# Autodesk Inventor assembly: Car_Assembly
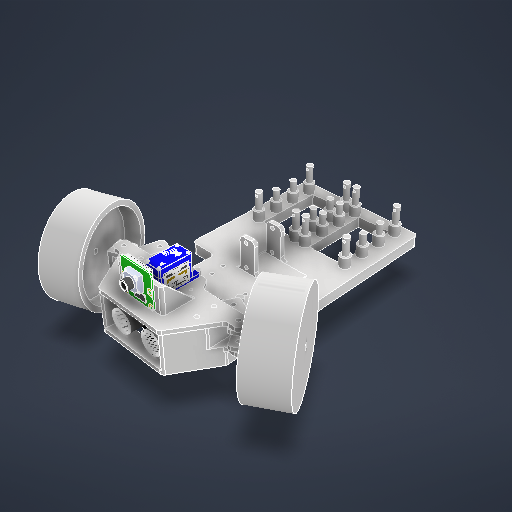
[picture p0: Inventor's stored thumbnail of the model, 512x512]
Saved by Autodesk Inventor 2025 (Build 290162000, 162)
## iProperties
Created: 2024-05-24
Part Number: Car_Assembly
Document SubType Name: Assembly
Designer: Garfieldcmix
Author: Garfieldcmix
## Documents named in this file (30)
- C:\Users\chaya\Desktop\WRO-2024-CAD\Inventor\Car_Assembly.iam
- C:\Users\chaya\Desktop\WRO-2024-CAD\Inventor\SG90 - Micro Servo 9g - Tower Pro\SG90 - Micro Servo 9g - Tower Pro.iam
- C:\Users\chaya\Desktop\WRO-2024-CAD\Inventor\Front_Bridge.ipt
- C:\Users\chaya\Desktop\WRO-2024-CAD\Inventor\Front_Wheel_Anchor.ipt
- C:\Users\chaya\Desktop\WRO-2024-CAD\Inventor\Front_Wheel_Anchor_MIR.ipt
- C:\Users\chaya\Desktop\WRO-2024-CAD\Inventor\Wheel.ipt
- C:\Users\chaya\Desktop\WRO-2024-CAD\Inventor\Wheel_MIR.ipt
- C:\Users\chaya\Desktop\WRO-2024-CAD\Inventor\Pi camera module3\Pi camera module3.ipt
- C:\Users\chaya\Desktop\WRO-2024-CAD\Inventor\4519 DkStone Technic Axle 3\4519 DkStone Technic Axle 3.ipt
- C:\Users\chaya\Desktop\WRO-2024-CAD\Inventor\Lego Beam Fram 5x7 (64179)\Lego Beam Fram 5x7 (64179).ipt
- C:\Users\chaya\Desktop\WRO-2024-CAD\Inventor\TT Motor\TT Motor.ipt
- C:\Users\chaya\Desktop\WRO-2024-CAD\Inventor\Lower_Chassis.ipt
- C:\Users\chaya\Desktop\WRO-2024-CAD\Inventor\Motor_Lego_Axle_Connector.ipt
- C:\Users\chaya\Desktop\WRO-2024-CAD\Inventor\Wheel_Lego_Axle_Connector.ipt
- C:\Users\chaya\Desktop\WRO-2024-CAD\Inventor\Front_Bridge_2.ipt
- C:\Users\chaya\Desktop\WRO-2024-CAD\Inventor\Servo_Steering_Linkage.ipt
- C:\Users\chaya\Desktop\WRO-2024-CAD\Inventor\hc-sr04\hc-sr04.iam
- C:\Users\chaya\Desktop\WRO-2024-CAD\Inventor\Lego_Frame_Holder.ipt
- C:\Users\chaya\Desktop\WRO-2024-CAD\Inventor\Lego_Frame_Holder_Extra.ipt
- C:\Users\chaya\Desktop\WRO-2024-CAD\Inventor\Lego_Frame_Holder_Extra_2.ipt
- C:\Users\chaya\Desktop\WRO-2024-CAD\Inventor\1.5_base.ipt
- C:\Users\chaya\Desktop\WRO-2024-CAD\Inventor\18650 2-WAY v5\18650 2-WAY v5.iam
- C:\Users\chaya\Desktop\WRO-2024-CAD\Inventor\MAKER-DRIVE\MAKER-DRIVE.iam
- C:\Users\chaya\Desktop\WRO-2024-CAD\Inventor\MPU_6050\MPU_6050.iam
- C:\Users\chaya\Desktop\WRO-2024-CAD\Inventor\RASPBERRY_PI_5\RASPBERRY_PI_5.iam
- C:\Users\chaya\Desktop\WRO-2024-CAD\Inventor\arduino nano\arduino nano.iam
- C:\Users\chaya\Desktop\WRO-2024-CAD\Inventor\Lego-Frame-Holder-Extra-Extra.ipt
- C:\Users\chaya\Desktop\WRO-2024-CAD\Inventor\SG90_Horn.ipt
- C:\Users\chaya\Desktop\WRO-2024-CAD\Inventor\2_Base.ipt
- C:\Users\chaya\Desktop\WRO-2024-CAD\Inventor\Wheel_Lego_Axle_Connector_2.ipt
## Components (54 placed, 37 different names)
1. Pi camera module3:1 — Mate:73, Mate:72, Mate:74
2. hc-sr04:1 [sub-assembly] — Mate:92, Mate:93, Mate:94
3. SG90_Servo [sub-assembly] — Mate:1, Mate:16, Mate:69, Mate:137, Mate:138
4. SG90_Horn:1 — Mate:137, Mate:138, Mate:139, Mate:141, Mate:201
5. Left_Servo_Steering_Linkage — Mate:85, Mate:83, Mate:139, Mate:141, Mate:202
6. Right_Servo_Steering_Linkage — Mate:199, Mate:200, Mate:201, Mate:202
7. Front_Bridge:1 — Mate:38, Mate:39, Mate:40, Mate:41, Mate:42, Mate:66, Mate:67, Mate:68, Mate:75, Mate:76, Mate:79, Mate:80, Angle:1, Mate:92, Mate:93, Mate:94
8. Front_Bridge_2:1 — Mate:66, Mate:67, Mate:68, Mate:69, Mate:73, Mate:72, Mate:74, Mate:1, Mate:16
9. Left_Front_Wheel_Anchor — Mate:75, Mate:76, Mate:77, Mate:78, Mate:85, Mate:83, Angle:1
10. Left_Front_Wheel — Mate:77, Mate:78
11. Right_Front_Wheel_Anchor — Mate:79, Mate:80, Mate:81, Mate:82, Mate:199, Mate:200
12. Right_Front_Wheel — Mate:81, Mate:82
13. Lower_Chassis:1 — Mate:38, Mate:39, Mate:40, Mate:41, Mate:42, Mate:43, Mate:44, Mate:45, Mate:46, Mate:47, Mate:48, Mate:57, Mate:91, Mate:96, Mate:97, Mate:98, Mate:100, Mate:101, Mate:103, Mate:104, Mate:106, Mate:107, Mate:109, Mate:110, Mate:112, Mate:113, Mate:115, Mate:116, Mate:118, Mate:119, Mate:120, Mate:121, Mate:122, Mate:123, Mate:124
14. Left_Lego_Beam_Frame — Mate:37, Mate:43, Mate:44, Mate:45, Mate:50, Mate:55, Mate:60, Mate:102, Mate:105, Mate:108, Mate:117
15. Lego_Driving_Shaft_Axle — Mate:50, Mate:53, Mate:54
16. TT Motor:1 — Mate:51, Mate:52, Mate:57, Mate:91
17. Motor_Lego_Axle_Connector — Mate:51, Mate:52, Mate:53, Mate:54, Mate:55
18. Right_Lego_Beam_Frame — Mate:46, Mate:47, Mate:48, Mate:49, Mate:63, Mate:95, Mate:99, Mate:111, Mate:114
19. Left_Lego_Wheel_Axle — Mate:37, Mate:58, Mate:59
20. Left_Wheel_Lego_Axle_Connector — Mate:58, Mate:59, Mate:60, Mate:219, Mate:220, Mate:221
21. Left_Wheel_Lego_Axle_Connector_2 — Mate:219, Mate:220, Mate:221, Mate:222, Mate:223
22. Left_Back_Wheel — Mate:222, Mate:223
23. Right_Lego_Wheel_Axle — Mate:49, Mate:61, Mate:62
24. Right_Wheel_Lego_Axle_Connector — Mate:61, Mate:62, Mate:63, Mate:224, Mate:225, Mate:226
25. Right_Wheel_Lego_Axle_Connector_2 — Mate:224, Mate:225, Mate:226, Mate:227, Mate:228
26. Right_Back_Wheel — Mate:227, Mate:228
27. Lego_Frame_Holder:1 — Mate:95, Mate:96, Mate:97
28. Lego_Frame_Holder:2 — Mate:98, Mate:99, Mate:100
29. Lego_Frame_Holder:3 — Mate:101, Mate:102, Mate:103
30. Lego_Frame_Holder:4 — Mate:104, Mate:105, Mate:106
31. Lego_Frame_Holder:5 — Mate:107, Mate:108, Mate:109
32. Lego_Frame_Holder:6 — Mate:110, Mate:111, Mate:112
33. Lego_Frame_Holder_Extra:1 — Mate:113, Mate:114, Mate:115, Mate:147, Mate:185, Mate:133, Mate:203
34. Lego_Frame_Holder_Extra:2 — Mate:116, Mate:117, Mate:118, Mate:125, Mate:128, Mate:187, Mate:188, Mate:204
35. Lego_Frame_Holder_Extra_2:1 — Mate:119, Mate:120, Mate:121, Mate:148, Mate:193, Mate:194, Mate:206
36. Lego_Frame_Holder_Extra_2:2 — Mate:122, Mate:123, Mate:124, Mate:126, Mate:149, Mate:191, Mate:192, Mate:205
37. 1.5_Base:1 — Mate:125, Mate:126, Mate:128, Mate:147, Mate:148, Mate:149, Mate:161, Mate:162, Mate:163, Mate:164, Mate:165, Mate:166, Mate:167, Mate:168, Mate:169, Mate:170, Mate:171, Mate:172, Mate:173, Mate:174, Mate:175, Mate:176, Mate:177, Mate:178, Mate:179, Mate:180, Mate:181, Mate:182, Mate:183, Mate:184
38. 18650 2-WAY v5:2 [sub-assembly] — Mate:164, Mate:165, Mate:166, Mate:167, Mate:173
39. hc-sr04:2 [sub-assembly] — Mate:179, Mate:180, Mate:181
40. hc-sr04:4 [sub-assembly] — Mate:182, Mate:183, Mate:184
41. hc-sr04:3 [sub-assembly] — Mate:174, Mate:175, Mate:176, Mate:177, Mate:178
42. MPU_6050:1 [sub-assembly] — Mate:161, Mate:162, Mate:163
43. arduino nano:1 [sub-assembly] — Mate:168, Mate:169, Mate:170, Mate:171, Mate:172
44. Lego-Frame-Holder-Extra-Extra:1 — Mate:185, Mate:133, Mate:146, Mate:186, Mate:203, Mate:216, Mate:218
45. Lego-Frame-Holder-Extra-Extra:2 — Mate:187, Mate:188, Mate:189, Mate:190, Mate:204, Mate:213, Mate:215
46. Lego-Frame-Holder-Extra-Extra:3 — Mate:191, Mate:192, Mate:195, Mate:196, Mate:205, Mate:210, Mate:212
47. Lego-Frame-Holder-Extra-Extra:4 — Mate:193, Mate:194, Mate:197, Mate:198, Mate:206, Mate:207, Mate:209
48. 2_Base:1 — Mate:146, Mate:151, Mate:152, Mate:153, Mate:154, Mate:155, Mate:156, Mate:157, Mate:158, Mate:159, Mate:160, Mate:186, Mate:189, Mate:190, Mate:195, Mate:196, Mate:197, Mate:198, Mate:208, Mate:211, Mate:214, Mate:217
49. RASPBERRY_PI_5:1 [sub-assembly] — Mate:151, Mate:152, Mate:153, Mate:154, Mate:155
50. MAKER-DRIVE:1 [sub-assembly] — Mate:156, Mate:157, Mate:158, Mate:159, Mate:160
51. Lego_Frame_Holder:7 — Mate:207, Mate:208, Mate:209
52. Lego_Frame_Holder:8 — Mate:210, Mate:211, Mate:212
53. Lego_Frame_Holder:9 — Mate:213, Mate:214, Mate:215
54. Lego_Frame_Holder:10 — Mate:216, Mate:217, Mate:218
## Relationships (170: Mate 169, Angle 1)
- Mate:1: SG90_Servo ↔ Front_Bridge_2:1
- Mate:16: SG90_Servo ↔ Front_Bridge_2:1
- Mate:37: Left_Lego_Beam_Frame ↔ Left_Lego_Wheel_Axle
- Mate:38: Front_Bridge:1 ↔ Lower_Chassis:1
- Mate:39: Front_Bridge:1 ↔ Lower_Chassis:1
- Mate:40: Front_Bridge:1 ↔ Lower_Chassis:1
- Mate:41: Front_Bridge:1 ↔ Lower_Chassis:1
- Mate:42: Front_Bridge:1 ↔ Lower_Chassis:1
- Mate:43: Lower_Chassis:1 ↔ Left_Lego_Beam_Frame
- Mate:44: Lower_Chassis:1 ↔ Left_Lego_Beam_Frame
- Mate:45: Lower_Chassis:1 ↔ Left_Lego_Beam_Frame
- Mate:46: Lower_Chassis:1 ↔ Right_Lego_Beam_Frame
- Mate:47: Lower_Chassis:1 ↔ Right_Lego_Beam_Frame
- Mate:48: Lower_Chassis:1 ↔ Right_Lego_Beam_Frame
- Mate:49: Right_Lego_Beam_Frame ↔ Right_Lego_Wheel_Axle
- Mate:50: Left_Lego_Beam_Frame ↔ Lego_Driving_Shaft_Axle
- Mate:51: TT Motor:1 ↔ Motor_Lego_Axle_Connector
- Mate:52: TT Motor:1 ↔ Motor_Lego_Axle_Connector
- Mate:53: Lego_Driving_Shaft_Axle ↔ Motor_Lego_Axle_Connector
- Mate:54: Lego_Driving_Shaft_Axle ↔ Motor_Lego_Axle_Connector
- Mate:55: Left_Lego_Beam_Frame ↔ Motor_Lego_Axle_Connector
- Mate:57: Lower_Chassis:1 ↔ TT Motor:1
- Mate:58: Left_Lego_Wheel_Axle ↔ Left_Wheel_Lego_Axle_Connector
- Mate:59: Left_Lego_Wheel_Axle ↔ Left_Wheel_Lego_Axle_Connector
- Mate:60: Left_Lego_Beam_Frame ↔ Left_Wheel_Lego_Axle_Connector
- Mate:61: Right_Lego_Wheel_Axle ↔ Right_Wheel_Lego_Axle_Connector
- Mate:62: Right_Lego_Wheel_Axle ↔ Right_Wheel_Lego_Axle_Connector
- Mate:63: Right_Lego_Beam_Frame ↔ Right_Wheel_Lego_Axle_Connector
- Mate:66: Front_Bridge:1 ↔ Front_Bridge_2:1
- Mate:67: Front_Bridge:1 ↔ Front_Bridge_2:1
- Mate:68: Front_Bridge:1 ↔ Front_Bridge_2:1
- Mate:69: SG90_Servo ↔ Front_Bridge_2:1
- Mate:73: Pi camera module3:1 ↔ Front_Bridge_2:1
- Mate:72: Pi camera module3:1 ↔ Front_Bridge_2:1
- Mate:74: Pi camera module3:1 ↔ Front_Bridge_2:1
- Mate:75: Front_Bridge:1 ↔ Left_Front_Wheel_Anchor
- Mate:76: Front_Bridge:1 ↔ Left_Front_Wheel_Anchor
- Mate:77: Left_Front_Wheel_Anchor ↔ Left_Front_Wheel
- Mate:78: Left_Front_Wheel_Anchor ↔ Left_Front_Wheel
- Mate:79: Front_Bridge:1 ↔ Right_Front_Wheel_Anchor
- Mate:80: Front_Bridge:1 ↔ Right_Front_Wheel_Anchor
- Mate:81: Right_Front_Wheel_Anchor ↔ Right_Front_Wheel
- Mate:82: Right_Front_Wheel_Anchor ↔ Right_Front_Wheel
- Mate:85: Left_Servo_Steering_Linkage ↔ Left_Front_Wheel_Anchor
- Mate:83: Left_Servo_Steering_Linkage ↔ Left_Front_Wheel_Anchor
- Angle:1 (180 deg): Front_Bridge:1 ↔ Left_Front_Wheel_Anchor
- Mate:91: Lower_Chassis:1 ↔ TT Motor:1
- Mate:92: hc-sr04:1 ↔ Front_Bridge:1
- Mate:93: hc-sr04:1 ↔ Front_Bridge:1
- Mate:94: hc-sr04:1 ↔ Front_Bridge:1
- Mate:95: Right_Lego_Beam_Frame ↔ Lego_Frame_Holder:1
- Mate:96: Lower_Chassis:1 ↔ Lego_Frame_Holder:1
- Mate:97: Lower_Chassis:1 ↔ Lego_Frame_Holder:1
- Mate:98: Lower_Chassis:1 ↔ Lego_Frame_Holder:2
- Mate:99: Right_Lego_Beam_Frame ↔ Lego_Frame_Holder:2
- Mate:100: Lower_Chassis:1 ↔ Lego_Frame_Holder:2
- Mate:101: Lower_Chassis:1 ↔ Lego_Frame_Holder:3
- Mate:102: Left_Lego_Beam_Frame ↔ Lego_Frame_Holder:3
- Mate:103: Lower_Chassis:1 ↔ Lego_Frame_Holder:3
- Mate:104: Lower_Chassis:1 ↔ Lego_Frame_Holder:4
- Mate:105: Left_Lego_Beam_Frame ↔ Lego_Frame_Holder:4
- Mate:106: Lower_Chassis:1 ↔ Lego_Frame_Holder:4
- Mate:107: Lower_Chassis:1 ↔ Lego_Frame_Holder:5
- Mate:108: Left_Lego_Beam_Frame ↔ Lego_Frame_Holder:5
- Mate:109: Lower_Chassis:1 ↔ Lego_Frame_Holder:5
- Mate:110: Lower_Chassis:1 ↔ Lego_Frame_Holder:6
- Mate:111: Right_Lego_Beam_Frame ↔ Lego_Frame_Holder:6
- Mate:112: Lower_Chassis:1 ↔ Lego_Frame_Holder:6
- Mate:113: Lower_Chassis:1 ↔ Lego_Frame_Holder_Extra:1
- Mate:114: Right_Lego_Beam_Frame ↔ Lego_Frame_Holder_Extra:1
- Mate:115: Lower_Chassis:1 ↔ Lego_Frame_Holder_Extra:1
- Mate:116: Lower_Chassis:1 ↔ Lego_Frame_Holder_Extra:2
- Mate:117: Left_Lego_Beam_Frame ↔ Lego_Frame_Holder_Extra:2
- Mate:118: Lower_Chassis:1 ↔ Lego_Frame_Holder_Extra:2
- Mate:119: Lower_Chassis:1 ↔ Lego_Frame_Holder_Extra_2:1
- Mate:120: Lower_Chassis:1 ↔ Lego_Frame_Holder_Extra_2:1
- Mate:121: Lower_Chassis:1 ↔ Lego_Frame_Holder_Extra_2:1
- Mate:122: Lower_Chassis:1 ↔ Lego_Frame_Holder_Extra_2:2
- Mate:123: Lower_Chassis:1 ↔ Lego_Frame_Holder_Extra_2:2
- Mate:124: Lower_Chassis:1 ↔ Lego_Frame_Holder_Extra_2:2
- Mate:125: Lego_Frame_Holder_Extra:2 ↔ 1.5_Base:1
- Mate:126: Lego_Frame_Holder_Extra_2:2 ↔ 1.5_Base:1
- Mate:185: Lego_Frame_Holder_Extra:1 ↔ Lego-Frame-Holder-Extra-Extra:1
- Mate:133: Lego_Frame_Holder_Extra:1 ↔ Lego-Frame-Holder-Extra-Extra:1
- Mate:128: Lego_Frame_Holder_Extra:2 ↔ 1.5_Base:1
- Mate:137: SG90_Servo ↔ SG90_Horn:1
- Mate:138: SG90_Servo ↔ SG90_Horn:1
- Mate:139: SG90_Horn:1 ↔ Left_Servo_Steering_Linkage
- Mate:141: SG90_Horn:1 ↔ Left_Servo_Steering_Linkage
- Mate:146: Lego-Frame-Holder-Extra-Extra:1 ↔ 2_Base:1
- Mate:147: Lego_Frame_Holder_Extra:1 ↔ 1.5_Base:1
- Mate:148: Lego_Frame_Holder_Extra_2:1 ↔ 1.5_Base:1
- Mate:149: Lego_Frame_Holder_Extra_2:2 ↔ 1.5_Base:1
- Mate:151: 2_Base:1 ↔ RASPBERRY_PI_5:1
- Mate:152: 2_Base:1 ↔ RASPBERRY_PI_5:1
- Mate:153: 2_Base:1 ↔ RASPBERRY_PI_5:1
- Mate:154: 2_Base:1 ↔ RASPBERRY_PI_5:1
- Mate:155: 2_Base:1 ↔ RASPBERRY_PI_5:1
- Mate:156: 2_Base:1 ↔ MAKER-DRIVE:1
- Mate:157: 2_Base:1 ↔ MAKER-DRIVE:1
- Mate:158: 2_Base:1 ↔ MAKER-DRIVE:1
- Mate:159: 2_Base:1 ↔ MAKER-DRIVE:1
- Mate:160: 2_Base:1 ↔ MAKER-DRIVE:1
- Mate:161: 1.5_Base:1 ↔ MPU_6050:1
- Mate:162: 1.5_Base:1 ↔ MPU_6050:1
- Mate:163: 1.5_Base:1 ↔ MPU_6050:1
- Mate:164: 1.5_Base:1 ↔ 18650 2-WAY v5:2
- Mate:165: 1.5_Base:1 ↔ 18650 2-WAY v5:2
- Mate:166: 1.5_Base:1 ↔ 18650 2-WAY v5:2
- Mate:167: 1.5_Base:1 ↔ 18650 2-WAY v5:2
- Mate:168: 1.5_Base:1 ↔ arduino nano:1
- Mate:169: 1.5_Base:1 ↔ arduino nano:1
- Mate:170: 1.5_Base:1 ↔ arduino nano:1
- Mate:171: 1.5_Base:1 ↔ arduino nano:1
- Mate:172: 1.5_Base:1 ↔ arduino nano:1
- Mate:173: 1.5_Base:1 ↔ 18650 2-WAY v5:2
- Mate:174: 1.5_Base:1 ↔ hc-sr04:3
- Mate:175: 1.5_Base:1 ↔ hc-sr04:3
- Mate:176: 1.5_Base:1 ↔ hc-sr04:3
- Mate:177: 1.5_Base:1 ↔ hc-sr04:3
- Mate:178: 1.5_Base:1 ↔ hc-sr04:3
- Mate:179: 1.5_Base:1 ↔ hc-sr04:2
- Mate:180: 1.5_Base:1 ↔ hc-sr04:2
- Mate:181: 1.5_Base:1 ↔ hc-sr04:2
- Mate:182: 1.5_Base:1 ↔ hc-sr04:4
- Mate:183: 1.5_Base:1 ↔ hc-sr04:4
- Mate:184: 1.5_Base:1 ↔ hc-sr04:4
- Mate:186: Lego-Frame-Holder-Extra-Extra:1 ↔ 2_Base:1
- Mate:187: Lego_Frame_Holder_Extra:2 ↔ Lego-Frame-Holder-Extra-Extra:2
- Mate:188: Lego_Frame_Holder_Extra:2 ↔ Lego-Frame-Holder-Extra-Extra:2
- Mate:189: Lego-Frame-Holder-Extra-Extra:2 ↔ 2_Base:1
- Mate:190: Lego-Frame-Holder-Extra-Extra:2 ↔ 2_Base:1
- Mate:191: Lego_Frame_Holder_Extra_2:2 ↔ Lego-Frame-Holder-Extra-Extra:3
- Mate:192: Lego_Frame_Holder_Extra_2:2 ↔ Lego-Frame-Holder-Extra-Extra:3
- Mate:193: Lego_Frame_Holder_Extra_2:1 ↔ Lego-Frame-Holder-Extra-Extra:4
- Mate:194: Lego_Frame_Holder_Extra_2:1 ↔ Lego-Frame-Holder-Extra-Extra:4
- Mate:195: Lego-Frame-Holder-Extra-Extra:3 ↔ 2_Base:1
- Mate:196: Lego-Frame-Holder-Extra-Extra:3 ↔ 2_Base:1
- Mate:197: Lego-Frame-Holder-Extra-Extra:4 ↔ 2_Base:1
- Mate:198: Lego-Frame-Holder-Extra-Extra:4 ↔ 2_Base:1
- Mate:199: Right_Servo_Steering_Linkage ↔ Right_Front_Wheel_Anchor
- Mate:200: Right_Servo_Steering_Linkage ↔ Right_Front_Wheel_Anchor
- Mate:201: SG90_Horn:1 ↔ Right_Servo_Steering_Linkage
- Mate:202: Left_Servo_Steering_Linkage ↔ Right_Servo_Steering_Linkage
- Mate:203: Lego_Frame_Holder_Extra:1 ↔ Lego-Frame-Holder-Extra-Extra:1
- Mate:204: Lego_Frame_Holder_Extra:2 ↔ Lego-Frame-Holder-Extra-Extra:2
- Mate:205: Lego_Frame_Holder_Extra_2:2 ↔ Lego-Frame-Holder-Extra-Extra:3
- Mate:206: Lego_Frame_Holder_Extra_2:1 ↔ Lego-Frame-Holder-Extra-Extra:4
- Mate:207: Lego-Frame-Holder-Extra-Extra:4 ↔ Lego_Frame_Holder:7
- Mate:208: 2_Base:1 ↔ Lego_Frame_Holder:7
- Mate:209: Lego-Frame-Holder-Extra-Extra:4 ↔ Lego_Frame_Holder:7
- Mate:210: Lego-Frame-Holder-Extra-Extra:3 ↔ Lego_Frame_Holder:8
- Mate:211: 2_Base:1 ↔ Lego_Frame_Holder:8
- Mate:212: Lego-Frame-Holder-Extra-Extra:3 ↔ Lego_Frame_Holder:8
- Mate:213: Lego-Frame-Holder-Extra-Extra:2 ↔ Lego_Frame_Holder:9
- Mate:214: 2_Base:1 ↔ Lego_Frame_Holder:9
- Mate:215: Lego-Frame-Holder-Extra-Extra:2 ↔ Lego_Frame_Holder:9
- Mate:216: Lego-Frame-Holder-Extra-Extra:1 ↔ Lego_Frame_Holder:10
- Mate:217: 2_Base:1 ↔ Lego_Frame_Holder:10
- Mate:218: Lego-Frame-Holder-Extra-Extra:1 ↔ Lego_Frame_Holder:10
- Mate:219: Left_Wheel_Lego_Axle_Connector ↔ Left_Wheel_Lego_Axle_Connector_2
- Mate:220: Left_Wheel_Lego_Axle_Connector ↔ Left_Wheel_Lego_Axle_Connector_2
- Mate:221: Left_Wheel_Lego_Axle_Connector ↔ Left_Wheel_Lego_Axle_Connector_2
- Mate:222: Left_Wheel_Lego_Axle_Connector_2 ↔ Left_Back_Wheel
- Mate:223: Left_Wheel_Lego_Axle_Connector_2 ↔ Left_Back_Wheel
- Mate:224: Right_Wheel_Lego_Axle_Connector ↔ Right_Wheel_Lego_Axle_Connector_2
- Mate:225: Right_Wheel_Lego_Axle_Connector ↔ Right_Wheel_Lego_Axle_Connector_2
- Mate:226: Right_Wheel_Lego_Axle_Connector ↔ Right_Wheel_Lego_Axle_Connector_2
- Mate:227: Right_Wheel_Lego_Axle_Connector_2 ↔ Right_Back_Wheel
- Mate:228: Right_Wheel_Lego_Axle_Connector_2 ↔ Right_Back_Wheel
